# Autodesk Inventor assembly: Base
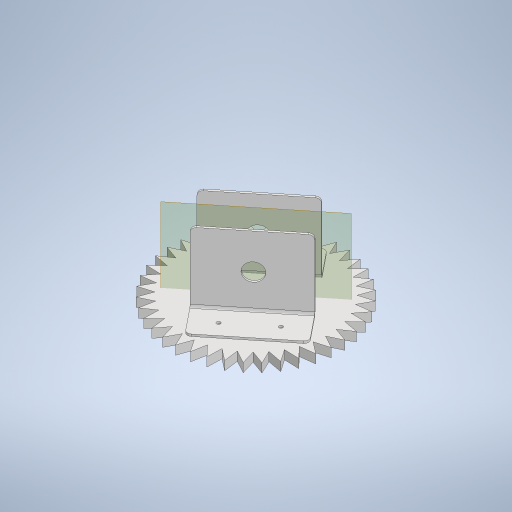
[picture p0: Inventor's stored thumbnail of the model, 512x512]
Saved by Autodesk Inventor 2023 (Build 270158030, 158C)
## iProperties
Created: 2022-10-06
Part Number: Base
Document SubType Name: Assembly
Designer: cjj5381
Author: cjj5381
## Documents named in this file (3)
- V:\Robtotics\Base\Base.iam
- V:\Robtotics\Base\BIG ASS GEAR.ipt
- V:\Robtotics\Base\Bracket.ipt
## Components (3 placed, 2 different names)
1. BIG ASS GEAR:1 — Mate:1, Mate:2, Flush:1, Mate:3, Mate:4, Mate:5, Mate:6, Mate:7, Mate:8
2. Bracket:1 — Mate:2, Mate:3, Mate:4
3. Bracket:2 — Mate:5, Mate:6, Mate:7, Angle:1
## Relationships (11: Mate 9, Flush 1, Angle 1)
- Mate:1: BIG ASS GEAR:1
- Mate:2: BIG ASS GEAR:1 ↔ Bracket:1
- Flush:1: BIG ASS GEAR:1
- Mate:3: BIG ASS GEAR:1 ↔ Bracket:1
- Mate:4: BIG ASS GEAR:1 ↔ Bracket:1
- Mate:5: BIG ASS GEAR:1 ↔ Bracket:2
- Mate:6: BIG ASS GEAR:1 ↔ Bracket:2
- Mate:7: BIG ASS GEAR:1 ↔ Bracket:2
- Mate:8: BIG ASS GEAR:1
- Mate:9
- Angle:1 (90 deg): Bracket:2
